# Autodesk Inventor assembly: 3899099 DHAS-MA-B6-80
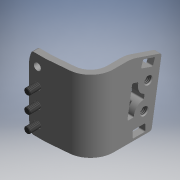
[picture p0: Inventor's stored thumbnail of the model, 180x180]
Saved by Autodesk Inventor 2017.3 (Build 213256000, 256)
## iProperties
Category: PARTsolutions
Company: FESTO
Part Number: 3899099 DHAS-MA-B6-80
Catalog Web Link: www.cadenas.de
Description: DHAS-MA-mounting bracket
Vendor: FESTO
Document SubType Name: Assembly
Designer: partserver
Manufacturer: FESTO
Mass: 38 g
Surface Area: 49.7069 cm^2
Volume: 5.65008 cm^3
Density: 6.72557 g/cm^3
Title: 3899099 DHAS-MA-B6-80
Author: Cadenas PARTsolutions
Comments: mounting bracket
PSOL_IDENT_0: {ATYP=ASSISTANT},{DATA=script=$CADENAS_DATA/23d-libs/festo/webfesto.vbb/&M_FAMILY=DHAS&M_GROUP=01&M_
PSOL_IDENT_1: PARTNO=3899099&IDCODE1=DHAS-MA-B6-80&IDCODE2=&customer_number_cns=&MATES=1&LOD=HI&LOCKERP=0&SINGLEPA
PSOL_IDENT_2: RT=1}
NB: 3899099 DHAS-MA-B6-80
NN: DHAS-MA
NT: mounting bracket
NBSYN: $TNR. $TYP.
LINA: 3899099 DHAS-MA-B6-80
CATALOG: Festo
TNR: 3899099
TYP: DHAS-MA-B6-80
CNSMASSEXACT: 0.038
SUPPLIER: FESTO
ARTICLENO: 3899099 DHAS-MA-B6-80
BOMINFO: 3899099 DHAS-MA-B6-80
CREATOR: CADENAS GmbH
## Documents named in this file (3)
- e:\temp\worker_61\temp\exporttempdir_7788_80_cjHSk\format_0\3899099 DHAS-MA-B6-80.iam
- e:\temp\worker_61\temp\exporttempdir_7788_80_cjHSk\format_0\3899099 DHAS-MA-B6-80---(winkel).ipt
- e:\temp\worker_61\temp\exporttempdir_7788_80_cjHSk\format_0\ISO-4762 M3x8.ipt
## Components (4 placed, 2 different names)
1. 3899099 DHAS-MA-B6-80---(winkel):1 — DIN912_1_XY@1 <-> ANBAU_XY@2, DIN912_1_Z@1 <-> ANBAU_Z@2, DIN912_1_YZ@1 <-> ANBAU_YZ@2, DIN912_2_XY@1 <-> ANBAU_XY@3, DIN912_2_Z@1 <-> ANBAU_Z@3, DIN912_2_YZ@1 <-> ANBAU_YZ@3, DIN912_3_XY@1 <-> ANBAU_XY@4, DIN912_3_Z@1 <-> ANBAU_Z@4, DIN912_3_YZ@1 <-> ANBAU_YZ@4
2. ISO-4762 M3x8:1 — DIN912_1_XY@1 <-> ANBAU_XY@2, DIN912_1_Z@1 <-> ANBAU_Z@2, DIN912_1_YZ@1 <-> ANBAU_YZ@2
3. ISO-4762 M3x8:2 — DIN912_2_XY@1 <-> ANBAU_XY@3, DIN912_2_Z@1 <-> ANBAU_Z@3, DIN912_2_YZ@1 <-> ANBAU_YZ@3
4. ISO-4762 M3x8:3 — DIN912_3_XY@1 <-> ANBAU_XY@4, DIN912_3_Z@1 <-> ANBAU_Z@4, DIN912_3_YZ@1 <-> ANBAU_YZ@4
## Relationships (9: Flush 3, Mate 3, Angle 3)
- DIN912_1_XY@1 <-> ANBAU_XY@2 [Flush]: 3899099 DHAS-MA-B6-80---(winkel):1 ↔ ISO-4762 M3x8:1
- DIN912_1_Z@1 <-> ANBAU_Z@2 [Mate]: 3899099 DHAS-MA-B6-80---(winkel):1 ↔ ISO-4762 M3x8:1
- DIN912_1_YZ@1 <-> ANBAU_YZ@2 [Angle] (0 deg): 3899099 DHAS-MA-B6-80---(winkel):1 ↔ ISO-4762 M3x8:1
- DIN912_2_XY@1 <-> ANBAU_XY@3 [Flush]: 3899099 DHAS-MA-B6-80---(winkel):1 ↔ ISO-4762 M3x8:2
- DIN912_2_Z@1 <-> ANBAU_Z@3 [Mate]: 3899099 DHAS-MA-B6-80---(winkel):1 ↔ ISO-4762 M3x8:2
- DIN912_2_YZ@1 <-> ANBAU_YZ@3 [Angle] (0 deg): 3899099 DHAS-MA-B6-80---(winkel):1 ↔ ISO-4762 M3x8:2
- DIN912_3_XY@1 <-> ANBAU_XY@4 [Flush]: 3899099 DHAS-MA-B6-80---(winkel):1 ↔ ISO-4762 M3x8:3
- DIN912_3_Z@1 <-> ANBAU_Z@4 [Mate]: 3899099 DHAS-MA-B6-80---(winkel):1 ↔ ISO-4762 M3x8:3
- DIN912_3_YZ@1 <-> ANBAU_YZ@4 [Angle] (0 deg): 3899099 DHAS-MA-B6-80---(winkel):1 ↔ ISO-4762 M3x8:3
